# Autodesk Inventor assembly: tete_prehension
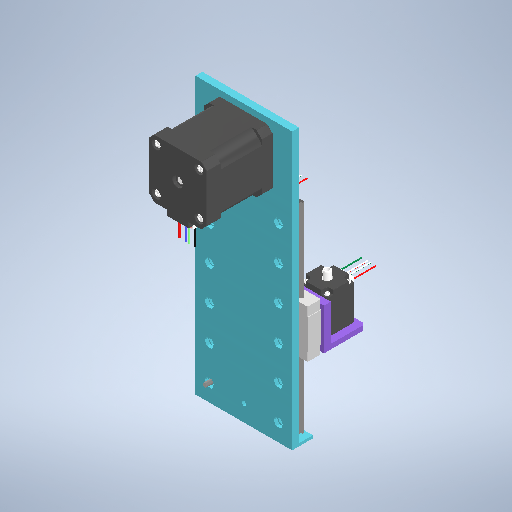
[picture p0: Inventor's stored thumbnail of the model, 512x512]
Saved by Autodesk Inventor 2025.1 (Build 291241000, 241)
## iProperties
Created: 2025-03-17
Part Number: tete_prehension
Document SubType Name: Assembly
Designer: felix
Author: felix
## Documents named in this file (8)
- D:\documents\projets inventor\Skibbidi Startech\tete_prehension.iam
- D:\documents\projets inventor\Skibbidi Startech\support_tete_prehension.ipt
- D:\documents\projets inventor\Skibbidi Startech\mgn12c_01.ipt
- C:\Users\felix\OneDrive - Haute Ecole de Namur-Liege-Luxembourg\Documents\Inventor\Content Center Files\R2025\fr-FR\BS EN ISO 4762\BS EN ISO 4762 - M3 x 12(1).ipt
- D:\documents\projets inventor\Skibbidi Startech\assemblage_nema8.iam
- D:\documents\projets inventor\Skibbidi Startech\assemblage_nema8_gauche.iam
- D:\documents\projets inventor\Skibbidi Startech\poulie courroie.ipt
- D:\documents\projets inventor\Skibbidi Startech\nema_17.ipt
## Components (10 placed, 7 different names)
1. support_tete_prehension:1 — Placage:2, Placage:3, Placage:4, Placage:5, Placage:6, Placage:7, Placage:10, Placage:11, Placage:12, Placage:13, Placage:14, Placage:15, Placage:21, Placage:22, Placage:23, Placage:24, Placage:25
2. mgn12c_01:1 — Placage:2, Placage:3, Placage:4, Placage:8, Placage:9, Placage:16
3. mgn12c_01:2 — Placage:5, Placage:6, Placage:7, Placage:17
4. BS EN ISO 4762 : Pièce 1 Vis cylindrique à six pans creux - Métrique M3 x 12:1 — Placage:8, Placage:9
5. mgn12c_01:3 — Placage:10, Placage:11, Placage:12, Placage:18, Placage:19
6. mgn12c_01:4 — Placage:13, Placage:14, Placage:15
7. assemblage_nema8:1 [sub-assembly] — Placage:16, Placage:17
8. assemblage_nema8_gauche:1 [sub-assembly] — Placage:18, Placage:19
9. poulie courroie:1 — Placage:21, Placage:22
10. nema_17:1 — Placage:23, Placage:24, Placage:25
## Relationships (23: Mate 23)
- Placage:2 [Mate]: support_tete_prehension:1 ↔ mgn12c_01:1
- Placage:3 [Mate]: support_tete_prehension:1 ↔ mgn12c_01:1
- Placage:4 [Mate]: support_tete_prehension:1 ↔ mgn12c_01:1
- Placage:5 [Mate]: support_tete_prehension:1 ↔ mgn12c_01:2
- Placage:6 [Mate]: support_tete_prehension:1 ↔ mgn12c_01:2
- Placage:7 [Mate]: support_tete_prehension:1 ↔ mgn12c_01:2
- Placage:8 [Mate]: mgn12c_01:1 ↔ BS EN ISO 4762 : Pièce 1 Vis cylindrique à six pans creux - Métrique M3 x 12:1
- Placage:9 [Mate]: mgn12c_01:1 ↔ BS EN ISO 4762 : Pièce 1 Vis cylindrique à six pans creux - Métrique M3 x 12:1
- Placage:10 [Mate]: support_tete_prehension:1 ↔ mgn12c_01:3
- Placage:11 [Mate]: support_tete_prehension:1 ↔ mgn12c_01:3
- Placage:12 [Mate]: support_tete_prehension:1 ↔ mgn12c_01:3
- Placage:13 [Mate]: support_tete_prehension:1 ↔ mgn12c_01:4
- Placage:14 [Mate]: support_tete_prehension:1 ↔ mgn12c_01:4
- Placage:15 [Mate]: support_tete_prehension:1 ↔ mgn12c_01:4
- Placage:16 [Mate]: mgn12c_01:1 ↔ assemblage_nema8:1
- Placage:17 [Mate]: mgn12c_01:2 ↔ assemblage_nema8:1
- Placage:18 [Mate]: mgn12c_01:3 ↔ assemblage_nema8_gauche:1
- Placage:19 [Mate]: mgn12c_01:3 ↔ assemblage_nema8_gauche:1
- Placage:21 [Mate]: support_tete_prehension:1 ↔ poulie courroie:1
- Placage:22 [Mate]: support_tete_prehension:1 ↔ poulie courroie:1
- Placage:23 [Mate]: support_tete_prehension:1 ↔ nema_17:1
- Placage:24 [Mate]: support_tete_prehension:1 ↔ nema_17:1
- Placage:25 [Mate]: support_tete_prehension:1 ↔ nema_17:1
